# Autodesk Inventor assembly: Ensamble_completo
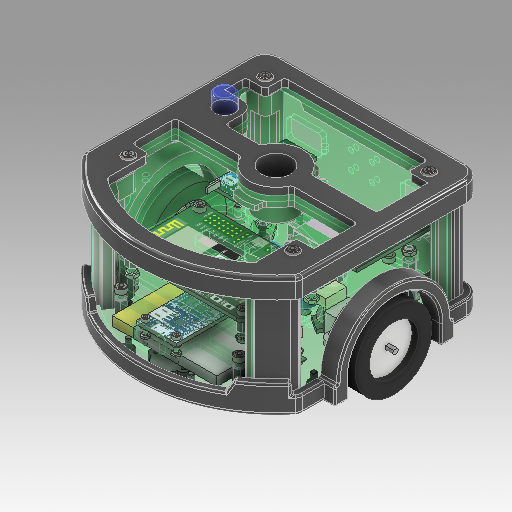
[picture p0: Inventor's stored thumbnail of the model, 512x512]
Saved by Autodesk Inventor 2027 (Build 310192000, 192)
## iProperties
Created: 2025-10-21
Part Number: Ensamble_completo
Document SubType Name: Assembly
Designer: brene
Author: brene
## Documents named in this file (46)
- C:\Users\06aar\OneDrive\Programas\GitHub\Atta-Bot-STEM\Chasis\Diseño V3.0\Ensamble_completo.iam
- C:\Users\06aar\OneDrive\Programas\GitHub\Atta-Bot-STEM\Chasis\Diseño V3.0\iParts\base_chasis_v6\base_chasis_v4-dimsAjustadas.ipt
- C:\Users\06aar\OneDrive\Programas\GitHub\Atta-Bot-STEM\Chasis\Diseño V3.0\base_chasis_v6.ipt
- C:\Users\06aar\OneDrive\Programas\GitHub\Atta-Bot-STEM\Chasis\Diseño V3.0\Content Center Files\en-US\ISO 4762(2)\ISO 4762 - M2 x 12ISO.ipt
- C:\Users\06aar\OneDrive\Programas\GitHub\Atta-Bot-STEM\Chasis\Diseño V3.0\switch.ipt
- C:\Users\06aar\OneDrive\Programas\GitHub\Atta-Bot-STEM\Chasis\Diseño V3.0\Content Center Files\en-US\ISO 4762(2)\ISO 4762 - M2 x 8ISO.ipt
- C:\Users\06aar\OneDrive\Programas\GitHub\Atta-Bot-STEM\Chasis\Diseño V3.0\Content Center Files\en-US\ISO 4032(2)\ISO 4032 - M2 - ISO.ipt
- C:\Users\06aar\OneDrive\Programas\GitHub\Atta-Bot-STEM\Chasis\Diseño V3.0\ball_caster.ipt
- C:\Users\06aar\OneDrive\Programas\GitHub\Atta-Bot-STEM\Chasis\Diseño V3.0\sensorInferior.ipt
- C:\Users\06aar\OneDrive\Programas\GitHub\Atta-Bot-STEM\Chasis\Diseño V3.0\Content Center Files\en-US\ISO 4762(2)\ISO 4762 - M3 x 12ISO.ipt
- C:\Users\06aar\OneDrive\Programas\GitHub\Atta-Bot-STEM\Chasis\Diseño V3.0\Content Center Files\en-US\ISO 4032(2)\ISO 4032 - M3 - ISO.ipt
- C:\Users\06aar\OneDrive\Programas\GitHub\Atta-Bot-STEM\Chasis\Diseño V3.0\spacers\hexagonal_spacer_MF_M3_H20_HEX5.5_FTD6_MTL6.ipt
- C:\Users\06aar\OneDrive\Programas\GitHub\Atta-Bot-STEM\Chasis\Diseño V3.0\spacers\hexagonal_spacer_MF_M3_H06_HEX5.5_FTD3_MTL6.ipt
- C:\Users\06aar\OneDrive\Programas\GitHub\Atta-Bot-STEM\Chasis\Diseño V3.0\Content Center Files\en-US\ISO 4762(2)\ISO 4762 - M3 x 8ISO.ipt
- C:\Users\06aar\OneDrive\Programas\GitHub\Atta-Bot-STEM\Chasis\Diseño V3.0\spacers\hexagonal_spacer_MF_M3_H08_HEX5_FTD4_MTL8.ipt
- C:\Users\06aar\OneDrive\Programas\GitHub\Atta-Bot-STEM\Chasis\Diseño V3.0\bateria.ipt
- C:\Users\06aar\OneDrive\Programas\GitHub\Atta-Bot-STEM\Chasis\Diseño V3.0\base_powerboost.ipt
- C:\Users\06aar\OneDrive\Programas\GitHub\Atta-Bot-STEM\Chasis\Diseño V3.0\powerboost.ipt
- C:\Users\06aar\OneDrive\Programas\GitHub\Atta-Bot-STEM\Chasis\Diseño V3.0\base_nivel2.ipt
- C:\Users\06aar\OneDrive\Programas\GitHub\Atta-Bot-STEM\Chasis\Diseño V3.0\ideaboard.ipt
- C:\Users\06aar\OneDrive\Programas\GitHub\Atta-Bot-STEM\Chasis\Diseño V3.0\sensorFrontal.ipt
- C:\Users\06aar\OneDrive\Programas\GitHub\Atta-Bot-STEM\Chasis\Diseño V3.0\Tower Pro MG90S Micro servo.ipt
- C:\Users\06aar\OneDrive\Programas\GitHub\Atta-Bot-STEM\Chasis\Diseño V3.0\spacers\hexagonal_spacer_MF_M3_H10_HEX5.5_FTD6_MTL6.ipt
- C:\Users\06aar\OneDrive\Programas\GitHub\Atta-Bot-STEM\Chasis\Diseño V3.0\SoporteMotor_3.0.ipt
- C:\Users\06aar\OneDrive\Programas\GitHub\Atta-Bot-STEM\Chasis\Diseño V3.0\motor.ipt
- C:\Users\06aar\OneDrive\Programas\GitHub\Atta-Bot-STEM\Chasis\Diseño V3.0\llanta.ipt
- C:\Users\06aar\OneDrive\Programas\GitHub\Atta-Bot-STEM\Chasis\Diseño V3.0\Unidirectional shoulder.ipt
- C:\Users\06aar\OneDrive\Programas\GitHub\Atta-Bot-STEM\Chasis\Diseño V3.0\SujecionServo.ipt
- C:\Users\06aar\OneDrive\Programas\GitHub\Atta-Bot-STEM\Chasis\Diseño V3.0\iParts\Esquinero Trasero\base_chasis_v4-dimsAjustadas.ipt
- C:\Users\06aar\OneDrive\Programas\GitHub\Atta-Bot-STEM\Chasis\Diseño V3.0\iParts\Bumper Trasero\base_chasis_v4-dimsAjustadas.ipt
- C:\Users\06aar\OneDrive\Programas\GitHub\Atta-Bot-STEM\Chasis\Diseño V3.0\Bumper Trasero.ipt
- C:\Users\06aar\OneDrive\Programas\GitHub\Atta-Bot-STEM\Chasis\Diseño V3.0\Guardabarros.ipt
- C:\Users\06aar\OneDrive\Programas\GitHub\Atta-Bot-STEM\Chasis\Diseño V3.0\Bumper Delantero.ipt
- C:\Users\06aar\OneDrive\Programas\GitHub\Atta-Bot-STEM\Chasis\Diseño V3.0\Esquineros Delanteros.ipt
- C:\Users\06aar\OneDrive\Programas\GitHub\Atta-Bot-STEM\Chasis\Diseño V3.0\PARED TRASERA.ipt
- C:\Users\06aar\OneDrive\Programas\GitHub\Atta-Bot-STEM\Chasis\Diseño V3.0\PAREDES LATERALES.ipt
- C:\Users\06aar\OneDrive\Programas\GitHub\Atta-Bot-STEM\Chasis\Diseño V3.0\PAREDES LATERALES_MIR.ipt
- C:\Users\06aar\OneDrive\Programas\GitHub\Atta-Bot-STEM\Chasis\Diseño V3.0\PARED FRONTAL.ipt
- C:\Users\06aar\OneDrive\Programas\GitHub\Atta-Bot-STEM\Chasis\Diseño V3.0\Techo Armadura.ipt
- C:\Users\06aar\OneDrive\Programas\GitHub\Atta-Bot-STEM\Chasis\Diseño V3.0\Acrilicos Superiores.ipt
- C:\Users\06aar\OneDrive\Programas\GitHub\Atta-Bot-STEM\Chasis\Diseño V3.0\Pieza de Silicona.ipt
- C:\Users\06aar\OneDrive\Programas\GitHub\Atta-Bot-STEM\Chasis\Diseño V3.0\PresaPilotInventorVersion.ipt
- C:\Users\06aar\OneDrive\Programas\GitHub\Atta-Bot-STEM\Chasis\Diseño V3.0\spacers\hexagonal_spacer_MF_M3_H20_HEX5.5_FTD6_MTL6_MIR.ipt
- C:\Users\06aar\OneDrive\Programas\GitHub\Atta-Bot-STEM\Chasis\Diseño V3.0\spacers\hexagonal_spacer_MF_M3_H06_HEX5.5_FTD3_MTL6_MIR.ipt
- C:\Users\06aar\OneDrive\Programas\GitHub\Atta-Bot-STEM\Chasis\Diseño V3.0\Esquinero Trasero.ipt
- C:\Users\06aar\OneDrive\Programas\GitHub\Atta-Bot-STEM\Chasis\Diseño V3.0\sensorInferior_MIR1.ipt
## Components (124 placed, 42 different names)
1. hexagonal_spacer_MF_M3_H06_HEX5.5_FTD3_MTL6_MIR:1 — Mate:312, Mate:314
2. hexagonal_spacer_MF_M3_H06_HEX5.5_FTD3_MTL6_MIR:2 — Mate:313, Mate:315
3. ISO 4032 M3:17 — Mate:313
4. ISO 4032 M3:18 — Mate:312
5. ISO 4762 M3 x 8:33 — Mate:315
6. ISO 4762 M3 x 8:34 — Mate:314
7. ISO 4762 M3 x 8:32
8. ISO 4762 M3 x 8:31
9. ISO 4762 M3 x 8:30 — Mate:310, Mate:311
10. ISO 4762 M3 x 8:29 — Mate:308, Mate:309
11. ISO 4762 M3 x 8:28 — Mate:304, Mate:305
12. ISO 4762 M3 x 8:27 — Mate:306, Mate:307
13. ISO 4762 M3 x 8:26
14. ISO 4762 M3 x 8:25
15. ISO 4762 M3 x 8:24
16. ISO 4762 M3 x 8:23
17. ISO 4762 M3 x 8:22
18. ISO 4762 M3 x 8:21
19. ISO 4762 M3 x 12:3
20. ISO 4762 M3 x 8:20 — Mate:301, Mate:302
21. ISO 4762 M3 x 8:19 — Mate:295, Mate:296
22. ISO 4762 M3 x 8:18 — Mate:299, Mate:300
23. ISO 4762 M3 x 8:17 — Mate:297, Mate:298
24. ISO 4762 M3 x 8:16 — Mate:293, Mate:294
25. ISO 4762 M3 x 8:15 — Mate:291, Mate:292
26. hexagonal_spacer_MF_M3_H20_HEX5.5_FTD6_MTL6:5 — Mate:289, Mate:290
27. hexagonal_spacer_MF_M3_H20_HEX5.5_FTD6_MTL6_MIR:1
28. ISO 4762 M3 x 8:10 — Mate:151, Mate:152
29. ISO 4762 M3 x 8:9 — Mate:153, Mate:154, Mate:285
30. hexagonal_spacer_MF_M3_H10_HEX5.5_FTD6_MTL6:2 — Mate:148, Mate:150
31. hexagonal_spacer_MF_M3_H10_HEX5.5_FTD6_MTL6:1 — Mate:147, Mate:149
32. ISO 4762 M3 x 8:8 — Mate:113, Mate:114, Mate:250, Mate:251
33. ISO 4762 M3 x 8:7 — Mate:117, Mate:118
34. ISO 4032 M3:8 — Mate:123, Mate:124
35. ISO 4032 M3:7 — Mate:125, Mate:126
36. hexagonal_spacer_MF_M3_H06_HEX5.5_FTD3_MTL6:10 — Mate:115, Mate:116, Mate:119, Mate:120, Mate:126
37. hexagonal_spacer_MF_M3_H06_HEX5.5_FTD3_MTL6:9 — Mate:111, Mate:112, Mate:121, Mate:122, Mate:124
38. hexagonal_spacer_MF_M3_H06_HEX5.5_FTD3_MTL6:8 — Mate:104, Mate:105, Mate:108, Mate:110, Mate:132, Mate:175
39. hexagonal_spacer_MF_M3_H06_HEX5.5_FTD3_MTL6:7 — Mate:106, Mate:107, Mate:134, Mate:177
40. ISO 4762 M3 x 8:6 — Mate:94, Mate:95
41. ISO 4762 M3 x 8:5 — Mate:96, Mate:97
42. ISO 4762 M3 x 8:4 — Mate:92, Mate:93
43. ISO 4762 M3 x 8:3 — Mate:98, Mate:99
44. ISO 4032 M2:9 — Mate:80, Mate:81
45. ISO 4032 M2:7 — Mate:82, Mate:83
46. ISO 4032 M2:6 — Mate:64, Mate:65, Mate:70
47. ISO 4032 M2:4 — Mate:62, Mate:63, Mate:71
48. ISO 4762 M2 x 12:2 — Mate:72, Mate:73, Mate:83
49. ISO 4762 M2 x 12:1 — Mate:74, Mate:75, Mate:81
50. ISO 4032 M3:6 — Mate:48, Mate:49, Mate:57
51. ISO 4032 M3:5 — Mate:50, Mate:51, Mate:59
52. ISO 4032 M3:4 — Mate:46, Mate:47, Mate:53
53. ISO 4032 M3:3 — Mate:44, Mate:45, Mate:55
54. hexagonal_spacer_MF_M3_H08_HEX5_FTD4_MTL8:4 — Mate:54, Mate:55, Mate:90
55. hexagonal_spacer_MF_M3_H08_HEX5_FTD4_MTL8:3 — Mate:52, Mate:53, Mate:89
56. hexagonal_spacer_MF_M3_H08_HEX5_FTD4_MTL8:2 — Mate:58, Mate:59, Mate:88
57. hexagonal_spacer_MF_M3_H08_HEX5_FTD4_MTL8:1 — Mate:56, Mate:57, Mate:61
58. ISO 4762 M3 x 8:2 — Mate:34, Mate:35, Mate:39
59. ISO 4762 M3 x 8:1 — Mate:32, Mate:33, Mate:37
60. hexagonal_spacer_MF_M3_H20_HEX5.5_FTD6_MTL6:4 — Mate:36, Mate:37, Mate:137, Mate:145
61. hexagonal_spacer_MF_M3_H20_HEX5.5_FTD6_MTL6:3 — Mate:38, Mate:39, Mate:143
62. hexagonal_spacer_MF_M3_H20_HEX5.5_FTD6_MTL6:2 — Mate:26, Mate:27, Mate:135, Mate:141
63. hexagonal_spacer_MF_M3_H20_HEX5.5_FTD6_MTL6:1 — Mate:24, Mate:25, Mate:136, Mate:139
64. ISO 4032 M3:2 — Mate:14, Mate:15, Mate:23
65. ISO 4032 M3:1 — Mate:12, Mate:13, Mate:21
66. ISO 4762 M3 x 12:2 — Mate:23, Mate:27
67. ISO 4762 M3 x 12:1 — Mate:21, Mate:25, Mate:283
68. ISO 4762 M2 x 8:4 — Mate:8, Mate:9, Tangent:4
69. ISO 4762 M2 x 8:3 — Mate:10, Mate:11, Tangent:3
70. ISO 4032 M2:2 — Insert:2
71. ISO 4032 M2:1 — Insert:1
72. ISO 4762 M2 x 8:2 — Mate:3, Mate:4
73. ISO 4762 M2 x 8:1 — Mate:5, Mate:6
74. ISO 4032 M3:16 — Mate:144, Mate:145
75. ISO 4032 M3:15 — Mate:140, Mate:141
76. ISO 4032 M3:14 — Mate:138, Mate:139
77. ISO 4032 M3:13 — Mate:142, Mate:143
78. ISO 4032 M3:11 — Mate:131, Mate:132
79. ISO 4032 M3:10 — Mate:129
80. ISO 4032 M3:9 — Mate:133, Mate:134
81. ISO 4032 M2:15 — Mate:194, Mate:195
82. ISO 4032 M2:14 — Mate:196, Mate:197
83. ISO 4032 M2:13 — Mate:192, Mate:193
84. ISO 4032 M2:12 — Mate:190, Mate:191
85. ISO 4762 M2 x 8:10 — Mate:183, Mate:197
86. ISO 4762 M2 x 8:9 — Mate:187, Mate:193
87. ISO 4762 M2 x 8:8 — Mate:189, Mate:191
88. ISO 4762 M2 x 8:7 — Mate:185, Mate:195
89. ISO 4762 M3 x 8:14 — Mate:174, Mate:175
90. ISO 4762 M3 x 8:11 — Mate:176, Mate:177
91. sensorInferior_MIR1:1
92. sensorInferior:3 — Mate:283, Mate:284
93. switch:1 — Mate:1, Mate:2, Mate:3, Mate:5, Angle:3
94. ball_caster:1 — Mate:7, Tangent:1, Tangent:2, Mate:9, Mate:11
95. bateria:1 — Mate:60, Mate:61, Mate:146, Angle:2
96. base_powerboost:1 — Mate:62, Mate:63, Mate:64, Mate:65, Mate:80, Mate:82, Mate:88, Mate:89, Mate:90, Mate:92, Mate:93, Mate:94, Mate:95, Mate:96, Mate:97, Mate:98, Mate:99
97. powerboost:1 — Mate:70, Mate:71, Mate:72, Mate:73, Mate:74, Mate:75
98. base_nivel2:1 — Mate:104, Mate:105, Mate:106, Mate:107, Mate:111, Mate:112, Mate:113, Mate:114, Mate:115, Mate:116, Mate:117, Mate:118, Mate:129, Mate:131, Mate:133, Mate:135, Mate:136, Mate:137, Mate:138, Mate:140, Mate:142, Mate:144, Angle:4, Angle:5, Mate:250, Mate:251
99. ideaboard:1 — Mate:108, Mate:110, Mate:174, Mate:176
100. sensorFrontal:1 — Mate:121, Mate:122, Mate:123, Angle:5
101. motor:1 — Mate:161, Mate:163, Mate:164, Mate:227, Tangent:5
102. sensorFrontal:2 — Mate:119, Mate:120, Mate:125, Angle:4
103. motor:2 — Mate:169, Mate:171, Mate:172, Mate:230, Tangent:6
104. llanta:1 — Mate:163, Mate:164, Mate:272
105. llanta:2 — Mate:171, Mate:172
106. Tower Pro MG90S Micro servo:2 — Mate:205, Mate:206, Mate:207, Mate:217
107. Unidirectional shoulder:1 — Mate:205, Mate:206
108. SujecionServo:1 — Mate:217
109. SoporteMotor_3.0:1 — Mate:229, Mate:230, Mate:231, Mate:233, Tangent:6
110. SoporteMotor_3.0:2 — Mate:226, Mate:227, Mate:228, Tangent:5, Mate:232
111. PARED TRASERA:1 — Mate:253, Mate:254
112. PAREDES LATERALES:2 — Mate:255, Mate:256, Mate:257
113. PAREDES LATERALES_MIR:1
114. PARED FRONTAL:1 — Mate:258, Mate:259, Mate:260, Mate:269
115. Acrilicos Superiores:1 — Mate:265, Mate:266, Mate:267
116. base_chasis_v6 — Mate:1, Mate:2, Mate:4, Mate:6, Insert:1, Insert:2, Mate:7, Tangent:1, Tangent:2, Mate:8, Mate:10, Tangent:3, Tangent:4, Mate:12, Mate:13, Mate:14, Mate:15, Mate:24, Mate:26, Mate:32, Mate:33, Mate:34, Mate:35, Mate:36, Mate:38, Mate:44, Mate:45, Mate:46, Mate:47, Mate:48, Mate:49, Mate:50, Mate:51, Mate:52, Mate:54, Mate:56, Mate:58, Mate:60, Mate:146, Mate:147, Mate:148, Mate:149, Mate:150, Mate:151, Mate:152, Mate:153, Mate:154, Mate:161, Mate:169, Mate:183, Mate:185, Mate:187, Mate:189, Mate:190, Mate:192, Mate:194, Mate:196, Mate:207, Mate:209, Flush:211, Mate:210, Angle:2, Angle:3, Mate:226, Mate:228, Mate:229, Mate:231, Mate:232, Mate:233, Flush:212, Mate:237, Mate:238, Mate:239, Mate:240, Mate:244, Mate:245, Mate:246, Mate:247, Mate:249, Mate:253, Mate:255, Mate:258, Mate:262, Mate:270, Mate:273, Mate:284, Mate:285, Mate:286, Mate:287, Mate:289, Mate:290, Mate:291, Mate:292, Mate:293, Mate:294, Mate:301, Mate:302
117. Esquinero Trasero — Flush:212, Mate:237, Mate:238, Mate:256, Mate:261, Mate:263, Mate:264
118. Bumper Trasero — Mate:239, Mate:240, Mate:244, Mate:254, Mate:304, Mate:305, Mate:306, Mate:307
119. Guardabarros:1 — Mate:270, Mate:272, Mate:273, Mate:295, Mate:296, Mate:297, Mate:298
120. Pieza de Silicona:1 — Flush:213, Mate:268
121. PresaPilotInventorVersion:1 — Mate:286, Mate:287, Mate:288
122. Bumper Delantero:1 — Mate:245, Mate:246, Mate:247, Mate:248, Mate:252, Mate:259, Mate:299, Mate:300
123. Esquineros Delanteros:1 — Mate:248, Mate:249, Mate:252, Mate:257, Mate:260, Mate:269
124. Techo Armadura:1 — Mate:261, Mate:262, Mate:263, Mate:264, Mate:265, Mate:266, Mate:267, Flush:213, Mate:268, Mate:308, Mate:309, Mate:310, Mate:311
## Relationships (235: Mate 220, Tangent 6, Angle 4, Flush 3, Insert 2)
- Mate:1: switch:1 ↔ base_chasis_v6
- Mate:2: switch:1 ↔ base_chasis_v6
- Mate:3: ISO 4762 M2 x 8:2 ↔ switch:1
- Mate:4: ISO 4762 M2 x 8:2 ↔ base_chasis_v6
- Mate:5: ISO 4762 M2 x 8:1 ↔ switch:1
- Mate:6: ISO 4762 M2 x 8:1 ↔ base_chasis_v6
- Insert:1: ISO 4032 M2:1 ↔ base_chasis_v6
- Insert:2: ISO 4032 M2:2 ↔ base_chasis_v6
- Mate:7: ball_caster:1 ↔ base_chasis_v6
- Tangent:1: ball_caster:1 ↔ base_chasis_v6
- Tangent:2: ball_caster:1 ↔ base_chasis_v6
- Mate:8: ISO 4762 M2 x 8:4 ↔ base_chasis_v6
- Mate:9: ISO 4762 M2 x 8:4 ↔ ball_caster:1
- Mate:10: ISO 4762 M2 x 8:3 ↔ base_chasis_v6
- Mate:11: ISO 4762 M2 x 8:3 ↔ ball_caster:1
- Tangent:3: ISO 4762 M2 x 8:3 ↔ base_chasis_v6
- Tangent:4: ISO 4762 M2 x 8:4 ↔ base_chasis_v6
- Mate:12: ISO 4032 M3:1 ↔ base_chasis_v6
- Mate:13: ISO 4032 M3:1 ↔ base_chasis_v6
- Mate:14: ISO 4032 M3:2 ↔ base_chasis_v6
- Mate:15: ISO 4032 M3:2 ↔ base_chasis_v6
- Mate:21: ISO 4032 M3:1 ↔ ISO 4762 M3 x 12:1
- Mate:23: ISO 4032 M3:2 ↔ ISO 4762 M3 x 12:2
- Mate:24: hexagonal_spacer_MF_M3_H20_HEX5.5_FTD6_MTL6:1 ↔ base_chasis_v6
- Mate:25: hexagonal_spacer_MF_M3_H20_HEX5.5_FTD6_MTL6:1 ↔ ISO 4762 M3 x 12:1
- Mate:26: hexagonal_spacer_MF_M3_H20_HEX5.5_FTD6_MTL6:2 ↔ base_chasis_v6
- Mate:27: hexagonal_spacer_MF_M3_H20_HEX5.5_FTD6_MTL6:2 ↔ ISO 4762 M3 x 12:2
- Mate:32: ISO 4762 M3 x 8:1 ↔ base_chasis_v6
- Mate:33: ISO 4762 M3 x 8:1 ↔ base_chasis_v6
- Mate:34: ISO 4762 M3 x 8:2 ↔ base_chasis_v6
- Mate:35: ISO 4762 M3 x 8:2 ↔ base_chasis_v6
- Mate:36: hexagonal_spacer_MF_M3_H20_HEX5.5_FTD6_MTL6:4 ↔ base_chasis_v6
- Mate:37: ISO 4762 M3 x 8:1 ↔ hexagonal_spacer_MF_M3_H20_HEX5.5_FTD6_MTL6:4
- Mate:38: hexagonal_spacer_MF_M3_H20_HEX5.5_FTD6_MTL6:3 ↔ base_chasis_v6
- Mate:39: ISO 4762 M3 x 8:2 ↔ hexagonal_spacer_MF_M3_H20_HEX5.5_FTD6_MTL6:3
- Mate:44: ISO 4032 M3:3 ↔ base_chasis_v6
- Mate:45: ISO 4032 M3:3 ↔ base_chasis_v6
- Mate:46: ISO 4032 M3:4 ↔ base_chasis_v6
- Mate:47: ISO 4032 M3:4 ↔ base_chasis_v6
- Mate:48: ISO 4032 M3:6 ↔ base_chasis_v6
- Mate:49: ISO 4032 M3:6 ↔ base_chasis_v6
- Mate:50: ISO 4032 M3:5 ↔ base_chasis_v6
- Mate:51: ISO 4032 M3:5 ↔ base_chasis_v6
- Mate:52: hexagonal_spacer_MF_M3_H08_HEX5_FTD4_MTL8:3 ↔ base_chasis_v6
- Mate:53: ISO 4032 M3:4 ↔ hexagonal_spacer_MF_M3_H08_HEX5_FTD4_MTL8:3
- Mate:54: hexagonal_spacer_MF_M3_H08_HEX5_FTD4_MTL8:4 ↔ base_chasis_v6
- Mate:55: ISO 4032 M3:3 ↔ hexagonal_spacer_MF_M3_H08_HEX5_FTD4_MTL8:4
- Mate:56: hexagonal_spacer_MF_M3_H08_HEX5_FTD4_MTL8:1 ↔ base_chasis_v6
- Mate:57: ISO 4032 M3:6 ↔ hexagonal_spacer_MF_M3_H08_HEX5_FTD4_MTL8:1
- Mate:58: hexagonal_spacer_MF_M3_H08_HEX5_FTD4_MTL8:2 ↔ base_chasis_v6
- Mate:59: ISO 4032 M3:5 ↔ hexagonal_spacer_MF_M3_H08_HEX5_FTD4_MTL8:2
- Mate:60: bateria:1 ↔ base_chasis_v6
- Mate:61: hexagonal_spacer_MF_M3_H08_HEX5_FTD4_MTL8:1 ↔ bateria:1
- Mate:62: ISO 4032 M2:4 ↔ base_powerboost:1
- Mate:63: ISO 4032 M2:4 ↔ base_powerboost:1
- Mate:64: ISO 4032 M2:6 ↔ base_powerboost:1
- Mate:65: ISO 4032 M2:6 ↔ base_powerboost:1
- Mate:70: ISO 4032 M2:6 ↔ powerboost:1
- Mate:71: ISO 4032 M2:4 ↔ powerboost:1
- Mate:72: ISO 4762 M2 x 12:2 ↔ powerboost:1
- Mate:73: ISO 4762 M2 x 12:2 ↔ powerboost:1
- Mate:74: ISO 4762 M2 x 12:1 ↔ powerboost:1
- Mate:75: ISO 4762 M2 x 12:1 ↔ powerboost:1
- Mate:80: ISO 4032 M2:9 ↔ base_powerboost:1
- Mate:81: ISO 4032 M2:9 ↔ ISO 4762 M2 x 12:1
- Mate:82: ISO 4032 M2:7 ↔ base_powerboost:1
- Mate:83: ISO 4032 M2:7 ↔ ISO 4762 M2 x 12:2
- Mate:88: hexagonal_spacer_MF_M3_H08_HEX5_FTD4_MTL8:2 ↔ base_powerboost:1
- Mate:89: hexagonal_spacer_MF_M3_H08_HEX5_FTD4_MTL8:3 ↔ base_powerboost:1
- Mate:90: hexagonal_spacer_MF_M3_H08_HEX5_FTD4_MTL8:4 ↔ base_powerboost:1
- Mate:92: ISO 4762 M3 x 8:4 ↔ base_powerboost:1
- Mate:93: ISO 4762 M3 x 8:4 ↔ base_powerboost:1
- Mate:94: ISO 4762 M3 x 8:6 ↔ base_powerboost:1
- Mate:95: ISO 4762 M3 x 8:6 ↔ base_powerboost:1
- Mate:96: ISO 4762 M3 x 8:5 ↔ base_powerboost:1
- Mate:97: ISO 4762 M3 x 8:5 ↔ base_powerboost:1
- Mate:98: ISO 4762 M3 x 8:3 ↔ base_powerboost:1
- Mate:99: ISO 4762 M3 x 8:3 ↔ base_powerboost:1
- Mate:104: hexagonal_spacer_MF_M3_H06_HEX5.5_FTD3_MTL6:8 ↔ base_nivel2:1
- Mate:105: hexagonal_spacer_MF_M3_H06_HEX5.5_FTD3_MTL6:8 ↔ base_nivel2:1
- Mate:106: hexagonal_spacer_MF_M3_H06_HEX5.5_FTD3_MTL6:7 ↔ base_nivel2:1
- Mate:107: hexagonal_spacer_MF_M3_H06_HEX5.5_FTD3_MTL6:7 ↔ base_nivel2:1
- Mate:108: hexagonal_spacer_MF_M3_H06_HEX5.5_FTD3_MTL6:8 ↔ ideaboard:1
- Mate:110: hexagonal_spacer_MF_M3_H06_HEX5.5_FTD3_MTL6:8 ↔ ideaboard:1
- Mate:111: hexagonal_spacer_MF_M3_H06_HEX5.5_FTD3_MTL6:9 ↔ base_nivel2:1
- Mate:112: hexagonal_spacer_MF_M3_H06_HEX5.5_FTD3_MTL6:9 ↔ base_nivel2:1
- Mate:113: ISO 4762 M3 x 8:8 ↔ base_nivel2:1
- Mate:114: ISO 4762 M3 x 8:8 ↔ base_nivel2:1
- Mate:115: hexagonal_spacer_MF_M3_H06_HEX5.5_FTD3_MTL6:10 ↔ base_nivel2:1
- Mate:116: hexagonal_spacer_MF_M3_H06_HEX5.5_FTD3_MTL6:10 ↔ base_nivel2:1
- Mate:117: ISO 4762 M3 x 8:7 ↔ base_nivel2:1
- Mate:118: ISO 4762 M3 x 8:7 ↔ base_nivel2:1
- Mate:119: hexagonal_spacer_MF_M3_H06_HEX5.5_FTD3_MTL6:10 ↔ sensorFrontal:2
- Mate:120: hexagonal_spacer_MF_M3_H06_HEX5.5_FTD3_MTL6:10 ↔ sensorFrontal:2
- Mate:121: hexagonal_spacer_MF_M3_H06_HEX5.5_FTD3_MTL6:9 ↔ sensorFrontal:1
- Mate:122: hexagonal_spacer_MF_M3_H06_HEX5.5_FTD3_MTL6:9 ↔ sensorFrontal:1
- Mate:123: ISO 4032 M3:8 ↔ sensorFrontal:1
- Mate:124: ISO 4032 M3:8 ↔ hexagonal_spacer_MF_M3_H06_HEX5.5_FTD3_MTL6:9
- Mate:125: ISO 4032 M3:7 ↔ sensorFrontal:2
- Mate:126: ISO 4032 M3:7 ↔ hexagonal_spacer_MF_M3_H06_HEX5.5_FTD3_MTL6:10
- Mate:129: ISO 4032 M3:10 ↔ base_nivel2:1
- Mate:131: ISO 4032 M3:11 ↔ base_nivel2:1
- Mate:132: hexagonal_spacer_MF_M3_H06_HEX5.5_FTD3_MTL6:8 ↔ ISO 4032 M3:11
- Mate:133: ISO 4032 M3:9 ↔ base_nivel2:1
- Mate:134: hexagonal_spacer_MF_M3_H06_HEX5.5_FTD3_MTL6:7 ↔ ISO 4032 M3:9
- Mate:135: hexagonal_spacer_MF_M3_H20_HEX5.5_FTD6_MTL6:2 ↔ base_nivel2:1
- Mate:136: hexagonal_spacer_MF_M3_H20_HEX5.5_FTD6_MTL6:1 ↔ base_nivel2:1
- Mate:137: hexagonal_spacer_MF_M3_H20_HEX5.5_FTD6_MTL6:4 ↔ base_nivel2:1
- Mate:138: ISO 4032 M3:14 ↔ base_nivel2:1
- Mate:139: hexagonal_spacer_MF_M3_H20_HEX5.5_FTD6_MTL6:1 ↔ ISO 4032 M3:14
- Mate:140: ISO 4032 M3:15 ↔ base_nivel2:1
- Mate:141: hexagonal_spacer_MF_M3_H20_HEX5.5_FTD6_MTL6:2 ↔ ISO 4032 M3:15
- Mate:142: ISO 4032 M3:13 ↔ base_nivel2:1
- Mate:143: hexagonal_spacer_MF_M3_H20_HEX5.5_FTD6_MTL6:3 ↔ ISO 4032 M3:13
- Mate:144: ISO 4032 M3:16 ↔ base_nivel2:1
- Mate:145: hexagonal_spacer_MF_M3_H20_HEX5.5_FTD6_MTL6:4 ↔ ISO 4032 M3:16
- Mate:146: bateria:1 ↔ base_chasis_v6
- Mate:147: hexagonal_spacer_MF_M3_H10_HEX5.5_FTD6_MTL6:1 ↔ base_chasis_v6
- Mate:148: hexagonal_spacer_MF_M3_H10_HEX5.5_FTD6_MTL6:2 ↔ base_chasis_v6
- Mate:149: hexagonal_spacer_MF_M3_H10_HEX5.5_FTD6_MTL6:1 ↔ base_chasis_v6
- Mate:150: hexagonal_spacer_MF_M3_H10_HEX5.5_FTD6_MTL6:2 ↔ base_chasis_v6
- Mate:151: ISO 4762 M3 x 8:10 ↔ base_chasis_v6
- Mate:152: ISO 4762 M3 x 8:10 ↔ base_chasis_v6
- Mate:153: ISO 4762 M3 x 8:9 ↔ base_chasis_v6
- Mate:154: ISO 4762 M3 x 8:9 ↔ base_chasis_v6
- Mate:161: motor:1 ↔ base_chasis_v6
- Mate:163: motor:1 ↔ llanta:1
- Mate:164: motor:1 ↔ llanta:1
- Mate:169: motor:2 ↔ base_chasis_v6
- Mate:171: motor:2 ↔ llanta:2
- Mate:172: motor:2 ↔ llanta:2
- Mate:174: ISO 4762 M3 x 8:14 ↔ ideaboard:1
- Mate:175: hexagonal_spacer_MF_M3_H06_HEX5.5_FTD3_MTL6:8 ↔ ISO 4762 M3 x 8:14
- Mate:176: ISO 4762 M3 x 8:11 ↔ ideaboard:1
- Mate:177: hexagonal_spacer_MF_M3_H06_HEX5.5_FTD3_MTL6:7 ↔ ISO 4762 M3 x 8:11
- Mate:183: ISO 4762 M2 x 8:10 ↔ base_chasis_v6
- Mate:185: ISO 4762 M2 x 8:7 ↔ base_chasis_v6
- Mate:187: ISO 4762 M2 x 8:9 ↔ base_chasis_v6
- Mate:189: ISO 4762 M2 x 8:8 ↔ base_chasis_v6
- Mate:190: ISO 4032 M2:12 ↔ base_chasis_v6
- Mate:191: ISO 4032 M2:12 ↔ ISO 4762 M2 x 8:8
- Mate:192: ISO 4032 M2:13 ↔ base_chasis_v6
- Mate:193: ISO 4032 M2:13 ↔ ISO 4762 M2 x 8:9
- Mate:194: ISO 4032 M2:15 ↔ base_chasis_v6
- Mate:195: ISO 4032 M2:15 ↔ ISO 4762 M2 x 8:7
- Mate:196: ISO 4032 M2:14 ↔ base_chasis_v6
- Mate:197: ISO 4032 M2:14 ↔ ISO 4762 M2 x 8:10
- Mate:205: Tower Pro MG90S Micro servo:2 ↔ Unidirectional shoulder:1
- Mate:206 (1 mm): Tower Pro MG90S Micro servo:2 ↔ Unidirectional shoulder:1
- Mate:207: Tower Pro MG90S Micro servo:2 ↔ base_chasis_v6
- Mate:209: base_chasis_v6
- Flush:211: base_chasis_v6
- Mate:210: base_chasis_v6
- Angle:2 (0 deg): bateria:1 ↔ base_chasis_v6
- Angle:3 (180 deg): switch:1 ↔ base_chasis_v6
- Angle:4 (180 deg): base_nivel2:1 ↔ sensorFrontal:2
- Angle:5 (180 deg): base_nivel2:1 ↔ sensorFrontal:1
- Mate:217: Tower Pro MG90S Micro servo:2 ↔ SujecionServo:1
- Mate:226: SoporteMotor_3.0:2 ↔ base_chasis_v6
- Mate:227: motor:1 ↔ SoporteMotor_3.0:2
- Mate:228: SoporteMotor_3.0:2 ↔ base_chasis_v6
- Mate:229: SoporteMotor_3.0:1 ↔ base_chasis_v6
- Mate:230: motor:2 ↔ SoporteMotor_3.0:1
- Mate:231: SoporteMotor_3.0:1 ↔ base_chasis_v6
- Tangent:5: motor:1 ↔ SoporteMotor_3.0:2
- Mate:232: SoporteMotor_3.0:2 ↔ base_chasis_v6
- Mate:233: SoporteMotor_3.0:1 ↔ base_chasis_v6
- Tangent:6: motor:2 ↔ SoporteMotor_3.0:1
- Flush:212: base_chasis_v6 ↔ Esquinero Trasero
- Mate:237: base_chasis_v6 ↔ Esquinero Trasero
- Mate:238: base_chasis_v6 ↔ Esquinero Trasero
- Mate:239: base_chasis_v6 ↔ Bumper Trasero
- Mate:240: base_chasis_v6 ↔ Bumper Trasero
- Mate:244: base_chasis_v6 ↔ Bumper Trasero
- Mate:245: base_chasis_v6 ↔ Bumper Delantero:1
- Mate:246: base_chasis_v6 ↔ Bumper Delantero:1
- Mate:247: base_chasis_v6 ↔ Bumper Delantero:1
- Mate:248: Bumper Delantero:1 ↔ Esquineros Delanteros:1
- Mate:249: base_chasis_v6 ↔ Esquineros Delanteros:1
- Mate:250: ISO 4762 M3 x 8:8 ↔ base_nivel2:1
- Mate:251: ISO 4762 M3 x 8:8 ↔ base_nivel2:1
- Mate:252: Bumper Delantero:1 ↔ Esquineros Delanteros:1
- Mate:253: PARED TRASERA:1 ↔ base_chasis_v6
- Mate:254: PARED TRASERA:1 ↔ Bumper Trasero
- Mate:255: PAREDES LATERALES:2 ↔ base_chasis_v6
- Mate:256: PAREDES LATERALES:2 ↔ Esquinero Trasero
- Mate:257: PAREDES LATERALES:2 ↔ Esquineros Delanteros:1
- Mate:258: PARED FRONTAL:1 ↔ base_chasis_v6
- Mate:259: PARED FRONTAL:1 ↔ Bumper Delantero:1
- Mate:260: PARED FRONTAL:1 ↔ Esquineros Delanteros:1
- Mate:261: Esquinero Trasero ↔ Techo Armadura:1
- Mate:262: base_chasis_v6 ↔ Techo Armadura:1
- Mate:263: Esquinero Trasero ↔ Techo Armadura:1
- Mate:264: Esquinero Trasero ↔ Techo Armadura:1
- Mate:265: Acrilicos Superiores:1 ↔ Techo Armadura:1
- Mate:266: Acrilicos Superiores:1 ↔ Techo Armadura:1
- Mate:267: Acrilicos Superiores:1 ↔ Techo Armadura:1
- Flush:213: Pieza de Silicona:1 ↔ Techo Armadura:1
- Mate:268: Pieza de Silicona:1 ↔ Techo Armadura:1
- Mate:269: PARED FRONTAL:1 ↔ Esquineros Delanteros:1
- Mate:270: base_chasis_v6 ↔ Guardabarros:1
- Mate:272: llanta:1 ↔ Guardabarros:1
- Mate:273: base_chasis_v6 ↔ Guardabarros:1
- Mate:283: ISO 4762 M3 x 12:1 ↔ sensorInferior:3
- Mate:284: sensorInferior:3 ↔ base_chasis_v6
- Mate:285: ISO 4762 M3 x 8:9 ↔ base_chasis_v6
- Mate:286: base_chasis_v6 ↔ PresaPilotInventorVersion:1
- Mate:287: base_chasis_v6 ↔ PresaPilotInventorVersion:1
- Mate:288: PresaPilotInventorVersion:1
- Mate:289: hexagonal_spacer_MF_M3_H20_HEX5.5_FTD6_MTL6:5 ↔ base_chasis_v6
- Mate:290: hexagonal_spacer_MF_M3_H20_HEX5.5_FTD6_MTL6:5 ↔ base_chasis_v6
- Mate:291: ISO 4762 M3 x 8:15 ↔ base_chasis_v6
- Mate:292: ISO 4762 M3 x 8:15 ↔ base_chasis_v6
- Mate:293: ISO 4762 M3 x 8:16 ↔ base_chasis_v6
- Mate:294: ISO 4762 M3 x 8:16 ↔ base_chasis_v6
- Mate:295: ISO 4762 M3 x 8:19 ↔ Guardabarros:1
- Mate:296: ISO 4762 M3 x 8:19 ↔ Guardabarros:1
- Mate:297: ISO 4762 M3 x 8:17 ↔ Guardabarros:1
- Mate:298: ISO 4762 M3 x 8:17 ↔ Guardabarros:1
- Mate:299: ISO 4762 M3 x 8:18 ↔ Bumper Delantero:1
- Mate:300: ISO 4762 M3 x 8:18 ↔ Bumper Delantero:1
- Mate:301: ISO 4762 M3 x 8:20 ↔ base_chasis_v6
- Mate:302: ISO 4762 M3 x 8:20 ↔ base_chasis_v6
- Mate:304: ISO 4762 M3 x 8:28 ↔ Bumper Trasero
- Mate:305: ISO 4762 M3 x 8:28 ↔ Bumper Trasero
- Mate:306: ISO 4762 M3 x 8:27 ↔ Bumper Trasero
- Mate:307: ISO 4762 M3 x 8:27 ↔ Bumper Trasero
- Mate:308: ISO 4762 M3 x 8:29 ↔ Techo Armadura:1
- Mate:309: ISO 4762 M3 x 8:29 ↔ Techo Armadura:1
- Mate:310: ISO 4762 M3 x 8:30 ↔ Techo Armadura:1
- Mate:311: ISO 4762 M3 x 8:30 ↔ Techo Armadura:1
- Mate:312: hexagonal_spacer_MF_M3_H06_HEX5.5_FTD3_MTL6_MIR:1 ↔ ISO 4032 M3:18
- Mate:313: hexagonal_spacer_MF_M3_H06_HEX5.5_FTD3_MTL6_MIR:2 ↔ ISO 4032 M3:17
- Mate:314: hexagonal_spacer_MF_M3_H06_HEX5.5_FTD3_MTL6_MIR:1 ↔ ISO 4762 M3 x 8:34
- Mate:315: hexagonal_spacer_MF_M3_H06_HEX5.5_FTD3_MTL6_MIR:2 ↔ ISO 4762 M3 x 8:33
